# Autodesk Inventor assembly: Structure
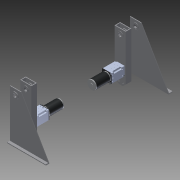
[picture p0: Inventor's stored thumbnail of the model, 180x180]
Saved by Autodesk Inventor 2013 (Build 170138000, 138)
## iProperties
Created: 2014-01-21
Part Number: Structure
Document SubType Name: Assembly
Designer: RobertB
Author: RobertB
## Documents named in this file (6)
- E:\Robotics\FRC\2014\CAD\Robot\Pickup\Structure.iam
- E:\Robotics\FRC\2014\CAD\Robot\Pickup\SuperStructure.ipt
- E:\Robotics\FRC\2014\CAD\Robot\Pickup\LPlate.ipt
- E:\Robotics\FRC\2014\CAD\Robot\Pickup\RPlate.ipt
- E:\Robotics\FRC\2014\CAD\Robot\Pickup\Bearing.ipt
- E:\Robotics\FRC\2014\CAD\Robot\Pickup\Imported Components\217-2 Stage Versaplanetary STEP\217-2 Stage Versaplanetary STEP.iam
## Components (12 placed, 5 different names)
1. SuperStructure:1 — Flush:1, Flush:2, Mate:1, Mate:2, Mate:3, Mate:4, Mate:5, Flush:3, Flush:6, Mate:14, Mate:16, Mate:17, Mate:18
2. SuperStructure:2 — Flush:1, Flush:2, Mate:1, Mate:6, Mate:7, Mate:8, Mate:9, Flush:4, Flush:5, Mate:15, Mate:19, Mate:20, Mate:21
3. LPlate:1 — Mate:12, Mate:13, Flush:4, Flush:5, Mate:15
4. RPlate:1 — Mate:10, Mate:11, Flush:3, Flush:6, Mate:14
5. Bearing:1 — Mate:12, Mate:13
6. Bearing:2 — Mate:7, Mate:9
7. Bearing:3 — Mate:6, Mate:8
8. Bearing:4 — Mate:2, Mate:4
9. Bearing:5 — Mate:10, Mate:11
10. Bearing:6 — Mate:3, Mate:5
11. 217-2 Stage Versaplanetary STEP:1 [sub-assembly] — Mate:19, Mate:20, Mate:21
12. 217-2 Stage Versaplanetary STEP:2 [sub-assembly] — Mate:16, Mate:17, Mate:18
## Relationships (27: Mate 21, Flush 6)
- Flush:1: SuperStructure:1 ↔ SuperStructure:2
- Flush:2: SuperStructure:1 ↔ SuperStructure:2
- Mate:1 (406.4 mm): SuperStructure:1 ↔ SuperStructure:2
- Mate:2: SuperStructure:1 ↔ Bearing:4
- Mate:3: SuperStructure:1 ↔ Bearing:6
- Mate:4: SuperStructure:1 ↔ Bearing:4
- Mate:5: SuperStructure:1 ↔ Bearing:6
- Mate:6: SuperStructure:2 ↔ Bearing:3
- Mate:7: SuperStructure:2 ↔ Bearing:2
- Mate:8: SuperStructure:2 ↔ Bearing:3
- Mate:9: SuperStructure:2 ↔ Bearing:2
- Mate:10: RPlate:1 ↔ Bearing:5
- Mate:11: RPlate:1 ↔ Bearing:5
- Mate:12: LPlate:1 ↔ Bearing:1
- Mate:13: LPlate:1 ↔ Bearing:1
- Flush:3: SuperStructure:1 ↔ RPlate:1
- Flush:4: SuperStructure:2 ↔ LPlate:1
- Flush:5: SuperStructure:2 ↔ LPlate:1
- Flush:6: SuperStructure:1 ↔ RPlate:1
- Mate:14 (44.45 mm): SuperStructure:1 ↔ RPlate:1
- Mate:15 (44.45 mm): SuperStructure:2 ↔ LPlate:1
- Mate:16: SuperStructure:1 ↔ 217-2 Stage Versaplanetary STEP:2
- Mate:17: SuperStructure:1 ↔ 217-2 Stage Versaplanetary STEP:2
- Mate:18: SuperStructure:1 ↔ 217-2 Stage Versaplanetary STEP:2
- Mate:19: SuperStructure:2 ↔ 217-2 Stage Versaplanetary STEP:1
- Mate:20: SuperStructure:2 ↔ 217-2 Stage Versaplanetary STEP:1
- Mate:21: SuperStructure:2 ↔ 217-2 Stage Versaplanetary STEP:1
